# Autodesk Inventor assembly: 03-3
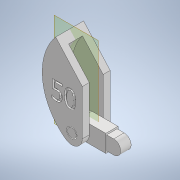
[picture p0: Inventor's stored thumbnail of the model, 180x180]
Saved by Autodesk Inventor 2022 (Build 260153000, 153)
## iProperties
Created: 2021-09-11
Part Number: 03-3
Document SubType Name: Assembly
Designer: 서울공업고등학교
Author: 서울공업고등학교
## Documents named in this file (3)
- C:\Users\서울공업고등학교\Documents\_9_11\3\03-3.iam
- C:\Users\서울공업고등학교\Documents\_9_11\3\03-1.ipt
- C:\Users\서울공업고등학교\Documents\_9_11\3\03-2.ipt
## Components (2 placed, 2 different names)
1. 03-1:1 — 메이트:1, 메이트:2
2. 03-2:1 — 메이트:1, 메이트:2
## Relationships (2: Mate 2)
- 메이트:1 [Mate] (0.5 mm): 03-1:1 ↔ 03-2:1
- 메이트:2 [Mate]: 03-1:1 ↔ 03-2:1
